# Autodesk Inventor assembly: Omni Wheel
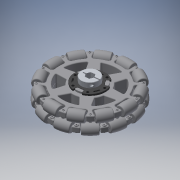
[picture p0: Inventor's stored thumbnail of the model, 180x180]
Saved by Autodesk Inventor 2019 (Build 230136000, 136)
## iProperties
Created: 2018-01-27
Part Number: Omni Wheel
Document SubType Name: Assembly
Designer: S-2512711
Author: S-2512711
## Documents named in this file (5)
- D:\Summer Drive Base V1\Summer Drivebase\Drivebase PowerUp Files\Omni Wheel.iam
- D:\Summer Drive Base V1\Summer Drivebase\Drivebase PowerUp Files\6_Omni-Directional_Wheel_217-2585.ipt
- D:\Summer Drive Base V1\Summer Drivebase\Drivebase PowerUp Files\1_2_Hex_Bore_Aluminum_VersaHub_217-2592.ipt
- D:\Summer Drive Base V1\Summer Drivebase\Drivebase PowerUp Files\1_2_Hex_Bore_Plastic_VersaHub_217-4009.ipt
- D:\Summer Drive Base V1\Summer Drivebase\am-1238+Collar+Clamp,+0.5''+Hex+Bore,+Aluminum.iam
## Components (4 placed, 4 different names)
1. 6_Omni-Directional_Wheel_217-2585:1 — Mate:1, Mate:2, Rotation:1, Mate:6, Mate:7, Mate:8, Mate:9
2. 1_2_Hex_Bore_Aluminum_VersaHub_217-2592:1 — Mate:7, Mate:8, Mate:9
3. 1_2_Hex_Bore_Plastic_VersaHub_217-4009:1 — Mate:1, Mate:2, Rotation:1, Mate:6, Mate:10, Flush:1, Flush:2
4. am-1238+Collar+Clamp,+0.5''+Hex+Bore,+Aluminum:1 [sub-assembly] — Mate:10, Flush:1, Flush:2
## Relationships (10: Mate 7, Flush 2, RelateRotation 1)
- Mate:1: 6_Omni-Directional_Wheel_217-2585:1 ↔ 1_2_Hex_Bore_Plastic_VersaHub_217-4009:1
- Mate:2: 6_Omni-Directional_Wheel_217-2585:1 ↔ 1_2_Hex_Bore_Plastic_VersaHub_217-4009:1
- Rotation:1 [RelateRotation] (1 ul): 6_Omni-Directional_Wheel_217-2585:1 ↔ 1_2_Hex_Bore_Plastic_VersaHub_217-4009:1
- Mate:6: 6_Omni-Directional_Wheel_217-2585:1 ↔ 1_2_Hex_Bore_Plastic_VersaHub_217-4009:1
- Mate:7: 6_Omni-Directional_Wheel_217-2585:1 ↔ 1_2_Hex_Bore_Aluminum_VersaHub_217-2592:1
- Mate:8: 6_Omni-Directional_Wheel_217-2585:1 ↔ 1_2_Hex_Bore_Aluminum_VersaHub_217-2592:1
- Mate:9: 6_Omni-Directional_Wheel_217-2585:1 ↔ 1_2_Hex_Bore_Aluminum_VersaHub_217-2592:1
- Mate:10: 1_2_Hex_Bore_Plastic_VersaHub_217-4009:1 ↔ am-1238+Collar+Clamp,+0.5''+Hex+Bore,+Aluminum:1
- Flush:1: 1_2_Hex_Bore_Plastic_VersaHub_217-4009:1 ↔ am-1238+Collar+Clamp,+0.5''+Hex+Bore,+Aluminum:1
- Flush:2: 1_2_Hex_Bore_Plastic_VersaHub_217-4009:1 ↔ am-1238+Collar+Clamp,+0.5''+Hex+Bore,+Aluminum:1
